# Autodesk Inventor assembly: pixyユニット
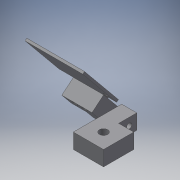
[picture p0: Inventor's stored thumbnail of the model, 180x180]
Saved by Autodesk Inventor 2017 (Build 210142000, 142)
## iProperties
Part Number: pixyユニット
Material: 一般
Document SubType Name: Assembly
Designer: highs
Author: highs
## Documents named in this file (4)
- C:\Users\highs\Desktop\学校\中の島\pixyユニット.iam
- C:\Users\highs\Desktop\学校\中の島\pixymount2.ipt
- C:\Users\highs\Desktop\学校\中の島\pixy.ipt
- C:\Users\highs\Desktop\学校\中の島\pixymount1.ipt
## Components (3 placed, 3 different names)
1. pixymount2:1 — メイト:1, メイト:6
2. pixy:1 — メイト:3, メイト:4, メイト:5
3. pixymount1:1 — メイト:1, メイト:3, メイト:4, メイト:5, メイト:6
## Relationships (5: Mate 5)
- メイト:1 [Mate]: pixymount2:1 ↔ pixymount1:1
- メイト:3 [Mate]: pixy:1 ↔ pixymount1:1
- メイト:4 [Mate]: pixy:1 ↔ pixymount1:1
- メイト:5 [Mate]: pixy:1 ↔ pixymount1:1
- メイト:6 [Mate]: pixymount2:1 ↔ pixymount1:1
